# Autodesk Inventor assembly: Gesamter_Zusammenbau
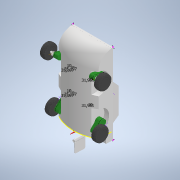
[picture p0: Inventor's stored thumbnail of the model, 180x180]
Saved by Autodesk Inventor 2021 (Build 250183000, 183)
## iProperties
Created: 2021-01-23
Part Number: Gesamter_Zusammenbau
Document SubType Name: Assembly
Designer: Jaro Machnow
Author: Jaro Machnow
## Documents named in this file (30)
- C:\Users\LETPJG\Documents\Vault\Gruppen\Gruppe 2\Entwurf\Amphibienfahrzeug\Gesamte Baugruppe\Gesamter_Zusammenbau.iam
- C:\Users\LETPJG\Documents\Vault\Gruppen\Gruppe 2\Entwurf\Amphibienfahrzeug\Gesamte Baugruppe\Karosserie.ipt
- C:\Users\LETPJG\Documents\Vault\Gruppen\Gruppe 2\Entwurf\Amphibienfahrzeug\Wechsel zwischen Land und Wasser\Mechanik_zum_Wechseln\Wechselmechnanik.iam
- C:\Users\LETPJG\Documents\Vault\Gruppen\Gruppe 2\Entwurf\Amphibienfahrzeug\Wechsel zwischen Land und Wasser\Wechselmechanik\Klappmechanismus2\Klapp-Baugruppe_vorn.iam
- C:\Users\LETPJG\Documents\Vault\Gruppen\Gruppe 2\Entwurf\Amphibienfahrzeug\Wechsel zwischen Land und Wasser\Wechselmechanik\Klappmechanismus\Klapp-Baugruppe_für_Antrieb.iam
- C:\Users\LETPJG\Documents\Vault\Gruppen\Gruppe 2\Entwurf\Amphibienfahrzeug\Karosserie\Karosserie\Karosserie_Abdeckung.ipt
- C:\Users\LETPJG\Documents\Vault\Gruppen\Gruppe 2\Entwurf\Amphibienfahrzeug\Rad.ipt
- C:\Users\LETPJG\Documents\Vault\Gruppen\Gruppe 2\Entwurf\Amphibienfahrzeug\Motor.ipt
- C:\Users\LETPJG\Documents\Vault\Gruppen\Gruppe 2\Entwurf\Amphibienfahrzeug\Planeten.iam
- C:\Users\LETPJG\Documents\Vault\Gruppen\Gruppe 2\Entwurf\Amphibienfahrzeug\radzuplanet.ipt
- C:\Users\LETPJG\Documents\Vault\Gruppen\Gruppe 2\Entwurf\Amphibienfahrzeug\motorzuplanete.ipt
- C:\Users\LETPJG\Documents\Vault\Gruppen\Gruppe 2\Entwurf\Amphibienfahrzeug\Wechselmotor.ipt
- C:\Users\LETPJG\Documents\Vault\Gruppen\Gruppe 2\Entwurf\Amphibienfahrzeug\Akku1.ipt
- C:\Users\LETPJG\Documents\Vault\Gruppen\Gruppe 2\Entwurf\Amphibienfahrzeug\Empfänger.ipt
- C:\Users\LETPJG\Documents\Vault\Gruppen\Gruppe 2\Entwurf\Amphibienfahrzeug\Steuereinheit.ipt
- C:\Users\LETPJG\Documents\Vault\Gruppen\Gruppe 2\Entwurf\Amphibienfahrzeug\Gesamte Baugruppe\Gesamter_Zusammenbau\AIP\Kabel und Kabelbaum\Gesamter_Zusammenbau.Kabelbaum4.iam
- C:\Users\LETPJG\Documents\Vault\Gruppen\Gruppe 2\Entwurf\Amphibienfahrzeug\RuderBauGruppe.iam
- C:\Users\LETPJG\Documents\Vault\Gruppen\Gruppe 2\Entwurf\Amphibienfahrzeug\SchiffsschraubeBaugruppe.ipt.iam
- C:\Users\LETPJG\Documents\Vault\Gruppen\Gruppe 2\Entwurf\Amphibienfahrzeug\Planeten\Konstruktions-Assistent\Kegelräder2.iam
- C:\Users\LETPJG\Documents\Vault\Gruppen\Gruppe 2\Entwurf\Amphibienfahrzeug\BauteilWelle7.ipt
- C:\Users\LETPJG\Documents\Vault\Gruppen\Gruppe 2\Entwurf\Amphibienfahrzeug\BauteilWelle2.ipt
- C:\Users\LETPJG\Documents\Vault\Gruppen\Gruppe 2\Entwurf\Amphibienfahrzeug\BauteilWelle8.ipt
- C:\Users\LETPJG\Documents\Vault\Gruppen\Gruppe 2\Entwurf\Amphibienfahrzeug\BauteilWelle9.ipt
- C:\Users\LETPJG\Documents\Vault\Gruppen\Gruppe 2\Entwurf\Amphibienfahrzeug\BauteilWelle3.ipt
- C:\Users\LETPJG\Documents\Vault\Gruppen\Gruppe 2\Entwurf\Amphibienfahrzeug\BauteilWelle4.ipt
- C:\Users\LETPJG\Documents\Inventor\Content Center Files\R2021\de-DE\ISO 10642(2)\ISO 10642  - M5  x  16.ipt
- C:\Users\LETPJG\Documents\Inventor\Content Center Files\R2021\de-DE\ISO 10642(2)\ISO 10642  - M5  x  8.ipt
- C:\Users\LETPJG\Documents\Vault\Gruppen\Gruppe 2\Entwurf\Amphibienfahrzeug\Wechsel zwischen Land und Wasser\Wechselmechanik\Klappmechanismus Antrieb.iam
- C:\Users\LETPJG\Documents\Vault\Gruppen\Gruppe 2\Entwurf\Amphibienfahrzeug\BauteilWelle15.ipt
- SchiffsschraubeBaugruppe.ipt
## Components (60 placed, 28 different names)
1. Karosserie:1 — Passend:17, Passend:18, Passend:19, Passend:20, Passend:21, Passend:22, Passend:23, Passend:24, Passend:25, Fluchtend:1, Fluchtend:2, Passend:63, Passend:67, Passend:75, Passend:76, Passend:77, Passend:78, Passend:80, Passend:81, Passend:82, Passend:97, Passend:98, Passend:109, Passend:110
2. Wechselmechnanik:1 [sub-assembly] — Passend:55, Passend:58, Passend:59, Passend:61, Passend:66, Passend:68, Passend:79, Drehbar:9, Winkel:1
3. Wechselmechnanik:2 [sub-assembly] — Passend:69, Passend:70, Passend:71, Passend:72, Drehbar:6, Passend:105, Passend:106, Passend:107, Passend:108
4. Klapp-Baugruppe_vorn:1 [sub-assembly] — Passend:17, Passend:18, Passend:31, Passend:36, Passend:39
5. Klapp-Baugruppe_vorn:2 [sub-assembly] — Passend:19, Passend:20, Passend:34, Passend:35, Passend:39
6. Klapp-Baugruppe_für_Antrieb:1 [sub-assembly] — Passend:21, Passend:22, Passend:32, Passend:37, Passend:38, Passend:45, Passend:46
7. Klapp-Baugruppe_für_Antrieb:2 [sub-assembly] — Passend:23, Passend:24, Passend:29, Passend:38, Passend:44, Passend:47, Passend:48, Passend:111
8. Karosserie_Abdeckung:1 — Passend:25, Fluchtend:1, Fluchtend:2
9. Rad:1 — Passend:29, Passend:111
10. Rad:2 — Passend:34, Passend:35
11. Rad:3 — Passend:32, Passend:37
12. Rad:4 — Passend:31, Passend:36
13. Motor:1 — Passend:63, Passend:64, Passend:65
14. Planeten:1 [sub-assembly] — Passend:44, Passend:55, Passend:58, Passend:62, Passend:79
15. radzuplanet:1 — Passend:45, Passend:46, Passend:62
16. radzuplanet:2 — Passend:47, Passend:48
17. Wechselmotor:1 — Passend:66, Passend:67, Passend:68
18. motorzuplanete:1 — Passend:59, Passend:61, Passend:64, Passend:65
19. Wechselmotor:2 — Passend:69, Passend:70, Passend:75, Passend:78
20. Motor:2 — Passend:73, Passend:74, Passend:76, Passend:77
21. motorzuplanete:2 — Passend:71, Passend:72, Passend:73, Passend:74
22. Akku1:2 — Passend:80
23. Empfänger:1 — Passend:81
24. Steuereinheit:1 — Passend:82
25. Kabelbaum4 [sub-assembly]
26. RuderBauGruppe:1 [sub-assembly] — Drehbar:1
27. SchiffsschraubeBaugruppe.ipt:1 [sub-assembly] — Einfügen:13
28. Kegelräder:1 [sub-assembly] — Drehbar:1, Einfügen:3
29. BauteilWelle7:1 — Einfügen:3, Drehbar:2
30. Kegelräder:2 [sub-assembly] — Drehbar:2, Einfügen:4
31. BauteilWelle2:1 — Einfügen:4, Drehbar:3
32. Kegelräder:3 [sub-assembly] — Drehbar:3, Einfügen:5
33. BauteilWelle7:2 — Einfügen:5, Drehbar:4
34. Kegelräder:4 [sub-assembly] — Drehbar:4, Einfügen:6
35. BauteilWelle8:1 — Einfügen:6, Drehbar:5
36. Kegelräder:5 [sub-assembly] — Drehbar:5, Einfügen:7
37. Kegelräder:6 [sub-assembly] — Drehbar:6, Passend:84
38. Kegelräder:7 [sub-assembly] — Drehbar:8, Passend:85, Passend:86
39. Kegelräder:8 [sub-assembly] — Drehbar:9, Einfügen:9
40. Kegelräder:9 [sub-assembly] — Passend:87, Passend:88, Passend:89, Passend:90
41. Kegelräder:10 [sub-assembly] — Einfügen:10, Einfügen:11
42. BauteilWelle9:1 — Einfügen:7, Passend:84
43. BauteilWelle2:2 — Drehbar:8, Einfügen:11
44. BauteilWelle3:1 — Passend:85, Passend:86, Passend:89, Passend:90
45. BauteilWelle4:1 — Einfügen:9, Winkel:1, Passend:87, Passend:88
46. Karosserie_Abdeckung:2 — Passend:97, Passend:98, Passend:99, Passend:100, Passend:101, Passend:102, Passend:103, Passend:104
47. DIN EN ISO 10642 M5  x  16:1 — Passend:99
48. DIN EN ISO 10642 M5  x  16:2 — Passend:100
49. DIN EN ISO 10642 M5  x  16:3 — Passend:101
50. DIN EN ISO 10642 M5  x  16:4 — Passend:102
51. DIN EN ISO 10642 M5  x  16:5 — Passend:103
52. DIN EN ISO 10642 M5  x  16:6 — Passend:104
53. DIN EN ISO 10642 M5  x  8:1 — Passend:105
54. DIN EN ISO 10642 M5  x  8:2 — Passend:106
55. DIN EN ISO 10642 M5  x  8:3 — Passend:107
56. DIN EN ISO 10642 M5  x  8:4 — Passend:108
57. Klappmechanismus Antrieb:1 [sub-assembly] — Passend:109
58. Klappmechanismus Antrieb:2 [sub-assembly] — Passend:110
59. BauteilWelle15:1 — Einfügen:10, Einfügen:12
60. Kegelräder:11 [sub-assembly] — Einfügen:12, Einfügen:13
## Relationships (91: Mate 70, Insert 10, RevoluteJoint 8, Flush 2, Angle 1)
- Passend:17 [Mate]: Karosserie:1 ↔ Klapp-Baugruppe_vorn:1
- Passend:18 [Mate] (3 mm): Karosserie:1 ↔ Klapp-Baugruppe_vorn:1
- Passend:19 [Mate]: Karosserie:1 ↔ Klapp-Baugruppe_vorn:2
- Passend:20 [Mate] (3 mm): Karosserie:1 ↔ Klapp-Baugruppe_vorn:2
- Passend:21 [Mate]: Karosserie:1 ↔ Klapp-Baugruppe_für_Antrieb:1
- Passend:22 [Mate] (3 mm): Karosserie:1 ↔ Klapp-Baugruppe_für_Antrieb:1
- Passend:23 [Mate]: Karosserie:1 ↔ Klapp-Baugruppe_für_Antrieb:2
- Passend:24 [Mate] (3 mm): Karosserie:1 ↔ Klapp-Baugruppe_für_Antrieb:2
- Passend:25 [Mate]: Karosserie:1 ↔ Karosserie_Abdeckung:1
- Fluchtend:1 [Flush]: Karosserie:1 ↔ Karosserie_Abdeckung:1
- Fluchtend:2 [Flush]: Karosserie:1 ↔ Karosserie_Abdeckung:1
- Passend:29 [Mate]: Klapp-Baugruppe_für_Antrieb:2 ↔ Rad:1
- Passend:31 [Mate]: Klapp-Baugruppe_vorn:1 ↔ Rad:4
- Passend:32 [Mate]: Klapp-Baugruppe_für_Antrieb:1 ↔ Rad:3
- Passend:34 [Mate]: Klapp-Baugruppe_vorn:2 ↔ Rad:2
- Passend:35 [Mate]: Klapp-Baugruppe_vorn:2 ↔ Rad:2
- Passend:36 [Mate]: Klapp-Baugruppe_vorn:1 ↔ Rad:4
- Passend:37 [Mate]: Klapp-Baugruppe_für_Antrieb:1 ↔ Rad:3
- Passend:38 [Mate]: Klapp-Baugruppe_für_Antrieb:1 ↔ Klapp-Baugruppe_für_Antrieb:2
- Passend:39 [Mate]: Klapp-Baugruppe_vorn:1 ↔ Klapp-Baugruppe_vorn:2
- Passend:44 [Mate]: Klapp-Baugruppe_für_Antrieb:2 ↔ Planeten:1
- Passend:45 [Mate]: Klapp-Baugruppe_für_Antrieb:1 ↔ radzuplanet:1
- Passend:46 [Mate]: Klapp-Baugruppe_für_Antrieb:1 ↔ radzuplanet:1
- Passend:47 [Mate]: Klapp-Baugruppe_für_Antrieb:2 ↔ radzuplanet:2
- Passend:48 [Mate]: Klapp-Baugruppe_für_Antrieb:2 ↔ radzuplanet:2
- Passend:55 [Mate]: Wechselmechnanik:1 ↔ Planeten:1
- Passend:58 [Mate]: Wechselmechnanik:1 ↔ Planeten:1
- Passend:59 [Mate]: Wechselmechnanik:1 ↔ motorzuplanete:1
- Passend:61 [Mate]: Wechselmechnanik:1 ↔ motorzuplanete:1
- Passend:62 [Mate]: Planeten:1 ↔ radzuplanet:1
- Passend:63 [Mate]: Karosserie:1 ↔ Motor:1
- Passend:64 [Mate]: Motor:1 ↔ motorzuplanete:1
- Passend:65 [Mate]: Motor:1 ↔ motorzuplanete:1
- Passend:66 [Mate]: Wechselmechnanik:1 ↔ Wechselmotor:1
- Passend:67 [Mate]: Karosserie:1 ↔ Wechselmotor:1
- Passend:68 [Mate]: Wechselmechnanik:1 ↔ Wechselmotor:1
- Passend:69 [Mate]: Wechselmechnanik:2 ↔ Wechselmotor:2
- Passend:70 [Mate]: Wechselmechnanik:2 ↔ Wechselmotor:2
- Passend:71 [Mate]: Wechselmechnanik:2 ↔ motorzuplanete:2
- Passend:72 [Mate]: Wechselmechnanik:2 ↔ motorzuplanete:2
- Passend:73 [Mate]: Motor:2 ↔ motorzuplanete:2
- Passend:74 [Mate]: Motor:2 ↔ motorzuplanete:2
- Passend:75 [Mate]: Karosserie:1 ↔ Wechselmotor:2
- Passend:76 [Mate]: Karosserie:1 ↔ Motor:2
- Passend:77 [Mate]: Karosserie:1 ↔ Motor:2
- Passend:78 [Mate]: Karosserie:1 ↔ Wechselmotor:2
- Passend:79 [Mate]: Wechselmechnanik:1 ↔ Planeten:1
- Passend:80 [Mate]: Karosserie:1 ↔ Akku1:2
- Passend:81 [Mate]: Karosserie:1 ↔ Empfänger:1
- Passend:82 [Mate]: Karosserie:1 ↔ Steuereinheit:1
- Drehbar:1 [RevoluteJoint]: RuderBauGruppe:1 ↔ Kegelräder:1
- Einfügen:3 [Insert]: Kegelräder:1 ↔ BauteilWelle7:1
- Drehbar:2 [RevoluteJoint]: BauteilWelle7:1 ↔ Kegelräder:2
- Einfügen:4 [Insert]: Kegelräder:2 ↔ BauteilWelle2:1
- Drehbar:3 [RevoluteJoint]: BauteilWelle2:1 ↔ Kegelräder:3
- Einfügen:5 [Insert]: Kegelräder:3 ↔ BauteilWelle7:2
- Drehbar:4 [RevoluteJoint]: BauteilWelle7:2 ↔ Kegelräder:4
- Einfügen:6 [Insert]: Kegelräder:4 ↔ BauteilWelle8:1
- Drehbar:5 [RevoluteJoint]: BauteilWelle8:1 ↔ Kegelräder:5
- Einfügen:7 [Insert]: Kegelräder:5 ↔ BauteilWelle9:1
- Drehbar:6 [RevoluteJoint]: Wechselmechnanik:2 ↔ Kegelräder:6
- Passend:84 [Mate]: Kegelräder:6 ↔ BauteilWelle9:1
- Drehbar:8 [RevoluteJoint]: Kegelräder:7 ↔ BauteilWelle2:2
- Passend:85 [Mate]: Kegelräder:7 ↔ BauteilWelle3:1
- Passend:86 [Mate]: Kegelräder:7 ↔ BauteilWelle3:1
- Drehbar:9 [RevoluteJoint]: Wechselmechnanik:1 ↔ Kegelräder:8
- Einfügen:9 [Insert]: Kegelräder:8 ↔ BauteilWelle4:1
- Winkel:1 [Angle] (90 deg): Wechselmechnanik:1 ↔ BauteilWelle4:1
- Passend:87 [Mate]: Kegelräder:9 ↔ BauteilWelle4:1
- Passend:88 [Mate]: Kegelräder:9 ↔ BauteilWelle4:1
- Passend:89 [Mate]: Kegelräder:9 ↔ BauteilWelle3:1
- Passend:90 [Mate]: Kegelräder:9 ↔ BauteilWelle3:1
- Passend:97 [Mate]: Karosserie:1 ↔ Karosserie_Abdeckung:2
- Passend:98 [Mate]: Karosserie:1 ↔ Karosserie_Abdeckung:2
- Passend:99 [Mate]: Karosserie_Abdeckung:2 ↔ DIN EN ISO 10642 M5  x  16:1
- Passend:100 [Mate]: Karosserie_Abdeckung:2 ↔ DIN EN ISO 10642 M5  x  16:2
- Passend:101 [Mate]: Karosserie_Abdeckung:2 ↔ DIN EN ISO 10642 M5  x  16:3
- Passend:102 [Mate]: Karosserie_Abdeckung:2 ↔ DIN EN ISO 10642 M5  x  16:4
- Passend:103 [Mate]: Karosserie_Abdeckung:2 ↔ DIN EN ISO 10642 M5  x  16:5
- Passend:104 [Mate]: Karosserie_Abdeckung:2 ↔ DIN EN ISO 10642 M5  x  16:6
- Passend:105 [Mate]: Wechselmechnanik:2 ↔ DIN EN ISO 10642 M5  x  8:1
- Passend:106 [Mate]: Wechselmechnanik:2 ↔ DIN EN ISO 10642 M5  x  8:2
- Passend:107 [Mate]: Wechselmechnanik:2 ↔ DIN EN ISO 10642 M5  x  8:3
- Passend:108 [Mate]: Wechselmechnanik:2 ↔ DIN EN ISO 10642 M5  x  8:4
- Passend:109 [Mate] (1 mm): Karosserie:1 ↔ Klappmechanismus Antrieb:1
- Passend:110 [Mate] (1 mm): Karosserie:1 ↔ Klappmechanismus Antrieb:2
- Einfügen:10 [Insert]: Kegelräder:10 ↔ BauteilWelle15:1
- Einfügen:11 [Insert]: Kegelräder:10 ↔ BauteilWelle2:2
- Einfügen:12 [Insert]: BauteilWelle15:1 ↔ Kegelräder:11
- Einfügen:13 [Insert]: SchiffsschraubeBaugruppe.ipt:1 ↔ Kegelräder:11
- Passend:111 [Mate] (-5 mm): Klapp-Baugruppe_für_Antrieb:2 ↔ Rad:1
